# Autodesk Inventor assembly: case
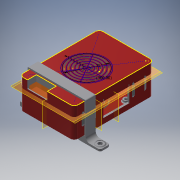
[picture p0: Inventor's stored thumbnail of the model, 180x180]
Saved by Autodesk Inventor 2019.3 (Build 233278000, 278)
## iProperties
Created: 2019-03-26
Part Number: case
Document SubType Name: Assembly
Designer: erwin
Author: erwin
## Documents named in this file (4)
- D:\GitHub\ElCheapoAIS-nmea\case\source\case.iam
- D:\GitHub\ElCheapoAIS-nmea\case\source\top_part.ipt
- D:\GitHub\ElCheapoAIS-nmea\case\source\bottom_part.ipt
- D:\GitHub\ElCheapoAIS-nmea\case\source\Imported Components\Arduino_DIN_rail_clip\Arduino_DIN_rail_clip.ipt
## Components (3 placed, 3 different names)
1. top_part:1
2. bottom_part:1 — Flush:2
3. Arduino_DIN_rail_clip:1 — Flush:2
## Relationships (1: Flush 1)
- Flush:2 (28 mm): bottom_part:1 ↔ Arduino_DIN_rail_clip:1
